# Autodesk Inventor assembly: ロボットベース
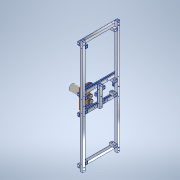
[picture p0: Inventor's stored thumbnail of the model, 180x180]
Saved by Autodesk Inventor 2020.3 (Build 243373000, 373)
## iProperties
Created: 2020-07-04
Part Number: ロボットベース
Document SubType Name: Assembly
Designer: totot
Mass: 783.518 g
Surface Area: 3392.37 cm^2
Volume: 312.689 cm^3
Density: 2.50574 g/cm^3
Author: totot
## Documents named in this file (12)
- D:\mysvn\ロボコン\キャチロボ\キャチロボ設計図\ロボット\ハンド\ロボットベース.iam
- D:\mysvn\ロボコン\キャチロボ\キャチロボ設計図\ロボット\ハンド\ロボットベース15x15_1.ipt
- D:\mysvn\ロボコン\キャチロボ\キャチロボ設計図\ロボット\ハンド\ロボットベース15x15_2.ipt
- D:\mysvn\ロボコン\キャチロボ\キャチロボ設計図\ロボット\ハンド\ロボットベース15x15x30.ipt
- D:\mysvn\ロボコン\キャチロボ\キャチロボ設計図\ロボット\ハンド\ロボットベース15x15x15.ipt
- D:\mysvn\ロボコン\キャチロボ\キャチロボ設計図\ロボット\ハンド\ロボットベース15x15_3.ipt
- D:\mysvn\ロボコン\キャチロボ\キャチロボ設計図\ロボット\ハンド\ロボットベース15x15_4.ipt
- D:\mysvn\ロボコン\キャチロボ\キャチロボ設計図\ロボット\ハンド\ロボットベース15x15_5.ipt
- D:\mysvn\ロボコン\キャチロボ\キャチロボ設計図\ロボット\ハンド\ロボットベースT5.5.ipt
- D:\mysvn\ロボコン\キャチロボ\キャチロボ設計図\ロボット\共有パーツ\RS_540.ipt
- D:\mysvn\ロボコン\キャチロボ\キャチロボ設計図\ロボット\共有パーツ\PS1-20_On.ipt
- D:\mysvn\ロボコン\キャチロボ\キャチロボ設計図\ロボット\共有パーツ\ポテンションメーター_BI-7284.ipt
## Components (26 placed, 11 different names)
1. ロボットベース15x15_1:2 — 挿入:2, 挿入:5, 挿入:7, 挿入:8, 挿入:32, 挿入:33
2. ロボットベース15x15_1:1 — 挿入:1, 挿入:3, 挿入:10, 挿入:12, 挿入:13, 挿入:14, 挿入:15, 挿入:16, 挿入:18
3. ロボットベース15x15_2:1 — 挿入:1, 挿入:2, 挿入:4, 挿入:6
4. ロボットベース15x15x30:1 — 挿入:3, 挿入:4
5. ロボットベース15x15x30:2 — 挿入:5, 挿入:6
6. ロボットベース15x15x30:3 — 挿入:8, 挿入:9
7. ロボットベース15x15x30:4 — 挿入:10, 挿入:11
8. ロボットベース15x15_2:2 — 挿入:7, 挿入:9, 挿入:11, 挿入:12
9. ロボットベース15x15_3:1 — 挿入:14, 挿入:17, 挿入:26, 挿入:27, 挿入:35, 挿入:36, 挿入:37
10. ロボットベース15x15x15:1 — 挿入:13
11. ロボットベース15x15x30:5 — 挿入:16, 挿入:19
12. ロボットベース15x15x30:6 — 挿入:15, 挿入:17
13. ロボットベース15x15_3:2 — 挿入:18, 挿入:19, 挿入:24, 挿入:28, 挿入:34, 挿入:38, 挿入:39
14. ロボットベース15x15x15:2 — 挿入:31
15. ロボットベース15x15x30:7 — 挿入:26, 挿入:30
16. ロボットベース15x15x30:8 — 挿入:24, 挿入:29
17. ロボットベース15x15_4:1 — 挿入:27, 挿入:28, 挿入:29, 挿入:30, 挿入:31
18. ロボットベース15x15x30:9 — 挿入:33, 挿入:35
19. ロボットベース15x15x30:10 — 挿入:32, 挿入:34
20. ロボットベース15x15_5:1 — 挿入:36, 挿入:37
21. ロボットベース15x15_5:2 — 挿入:38, 挿入:39
22. ロボットベースT5.5:1 — 挿入:42, 挿入:43, 挿入:44
23. RS_540:1 — 挿入:42, 挿入:43, 正接:1, フラッシュ:1
24. PS1-20_On:1 — 正接:1, フラッシュ:1
25. ポテンションメーター_BI-7284:1 — 挿入:44, 挿入:45
26. PS1-20_On:2 — 挿入:45
## Relationships (42: Insert 40, Tangent 1, Flush 1)
- 挿入:1 [Insert]: ロボットベース15x15_1:1 ↔ ロボットベース15x15_2:1
- 挿入:2 [Insert]: ロボットベース15x15_1:2 ↔ ロボットベース15x15_2:1
- 挿入:3 [Insert]: ロボットベース15x15_1:1 ↔ ロボットベース15x15x30:1
- 挿入:4 [Insert]: ロボットベース15x15_2:1 ↔ ロボットベース15x15x30:1
- 挿入:5 [Insert]: ロボットベース15x15_1:2 ↔ ロボットベース15x15x30:2
- 挿入:6 [Insert]: ロボットベース15x15_2:1 ↔ ロボットベース15x15x30:2
- 挿入:7 [Insert]: ロボットベース15x15_1:2 ↔ ロボットベース15x15_2:2
- 挿入:8 [Insert]: ロボットベース15x15_1:2 ↔ ロボットベース15x15x30:3
- 挿入:9 [Insert]: ロボットベース15x15x30:3 ↔ ロボットベース15x15_2:2
- 挿入:10 [Insert]: ロボットベース15x15_1:1 ↔ ロボットベース15x15x30:4
- 挿入:11 [Insert]: ロボットベース15x15x30:4 ↔ ロボットベース15x15_2:2
- 挿入:12 [Insert]: ロボットベース15x15_1:1 ↔ ロボットベース15x15_2:2
- 挿入:13 [Insert]: ロボットベース15x15_1:1 ↔ ロボットベース15x15x15:1
- 挿入:14 [Insert]: ロボットベース15x15_1:1 ↔ ロボットベース15x15_3:1
- 挿入:15 [Insert]: ロボットベース15x15_1:1 ↔ ロボットベース15x15x30:6
- 挿入:16 [Insert]: ロボットベース15x15_1:1 ↔ ロボットベース15x15x30:5
- 挿入:17 [Insert]: ロボットベース15x15_3:1 ↔ ロボットベース15x15x30:6
- 挿入:18 [Insert]: ロボットベース15x15_1:1 ↔ ロボットベース15x15_3:2
- 挿入:19 [Insert]: ロボットベース15x15x30:5 ↔ ロボットベース15x15_3:2
- 挿入:24 [Insert]: ロボットベース15x15_3:2 ↔ ロボットベース15x15x30:8
- 挿入:26 [Insert]: ロボットベース15x15_3:1 ↔ ロボットベース15x15x30:7
- 挿入:27 [Insert]: ロボットベース15x15_3:1 ↔ ロボットベース15x15_4:1
- 挿入:28 [Insert]: ロボットベース15x15_3:2 ↔ ロボットベース15x15_4:1
- 挿入:29 [Insert]: ロボットベース15x15x30:8 ↔ ロボットベース15x15_4:1
- 挿入:30 [Insert]: ロボットベース15x15x30:7 ↔ ロボットベース15x15_4:1
- 挿入:31 [Insert]: ロボットベース15x15x15:2 ↔ ロボットベース15x15_4:1
- 挿入:32 [Insert]: ロボットベース15x15_1:2 ↔ ロボットベース15x15x30:10
- 挿入:33 [Insert]: ロボットベース15x15_1:2 ↔ ロボットベース15x15x30:9
- 挿入:34 [Insert]: ロボットベース15x15_3:2 ↔ ロボットベース15x15x30:10
- 挿入:35 [Insert]: ロボットベース15x15_3:1 ↔ ロボットベース15x15x30:9
- 挿入:36 [Insert]: ロボットベース15x15_3:1 ↔ ロボットベース15x15_5:1
- 挿入:37 [Insert]: ロボットベース15x15_3:1 ↔ ロボットベース15x15_5:1
- 挿入:38 [Insert]: ロボットベース15x15_3:2 ↔ ロボットベース15x15_5:2
- 挿入:39 [Insert]: ロボットベース15x15_3:2 ↔ ロボットベース15x15_5:2
- [Insert]: ロボットベース15x15_5:2 ↔ ロボットベースT5.5:1
- [Insert]: ロボットベース15x15_5:2 ↔ ロボットベースT5.5:1
- 挿入:42 [Insert]: ロボットベースT5.5:1 ↔ RS_540:1
- 挿入:43 [Insert]: ロボットベースT5.5:1 ↔ RS_540:1
- 正接:1 [Tangent]: RS_540:1 ↔ PS1-20_On:1
- フラッシュ:1 [Flush]: RS_540:1 ↔ PS1-20_On:1
- 挿入:44 [Insert]: ロボットベースT5.5:1 ↔ ポテンションメーター_BI-7284:1
- 挿入:45 [Insert]: ポテンションメーター_BI-7284:1 ↔ PS1-20_On:2
## Named parameters: d39_d2 = 0 mm, d40_d3 = 0 mm
